# Autodesk Inventor assembly: GI - 100
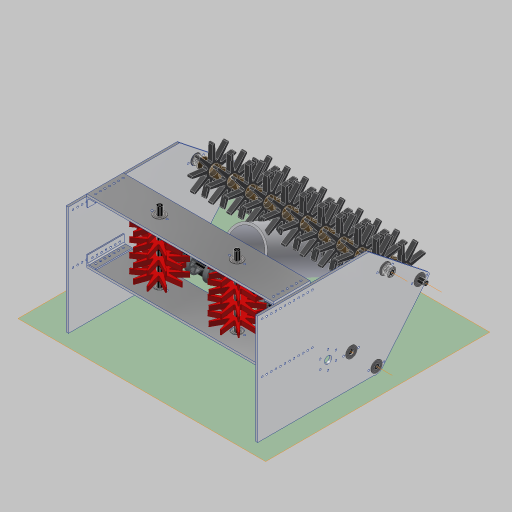
[picture p0: Inventor's stored thumbnail of the model, 512x512]
Saved by Autodesk Inventor 2023.5 (Build 275446000, 446)
## iProperties
Created: 2025-01-18
Part Number: GI - 100
Document SubType Name: Assembly
Designer: mavericks
Mass: 7269.96 g
Surface Area: 17734.9 cm^2
Volume: 4192.4 cm^3
Density: 1.73408 g/cm^3
Author: mavericks
## Documents named in this file (17)
- C:\Users\slick\OneDrive\Desktop\2025-ReefScape---CAD\ground intake\GI - 100.iam
- C:\Users\slick\OneDrive\Desktop\2025-ReefScape---CAD\ground intake\GI1\GI - 001.ipt
- C:\Users\slick\OneDrive\Desktop\2025-ReefScape---CAD\COMMON PARTS\BEARINGS\13_75mm_1_2_ThunderHex_ID_x_1_125_OD_x_0_313_WD_Flanged_Bearing_217-4006_MIR.ipt
- C:\Users\slick\OneDrive\Desktop\2025-ReefScape---CAD\ground intake\GI1\GI - 002.ipt
- C:\Users\slick\OneDrive\Desktop\2025-ReefScape---CAD\COMMON PARTS\WHEELS\2_OD_Straight_Flex_Wheel_217-6354.ipt
- C:\Users\slick\OneDrive\Desktop\2025-ReefScape---CAD\ground intake\GI - 200.iam
- C:\Users\slick\OneDrive\Desktop\2025-ReefScape---CAD\COMMON PARTS\MOTORS\Kracken with Cover and Boards.iam
- C:\Users\slick\OneDrive\Desktop\2025-ReefScape---CAD\COMMON PARTS\PULLEYS\gt2\16T Gt2 Kracken PullyWCP-1178.ipt
- C:\Users\slick\OneDrive\Desktop\2025-ReefScape---CAD\COMMON PARTS\PULLEYS\gt2\24t_x_9mm_Wide_Double_Flange_Aluminum_Pulley_GT2_3mm_1_2_Hex_Bore_217-5875.ipt
- C:\Users\slick\OneDrive\Desktop\2025-ReefScape---CAD\COMMON PARTS\PULLEYS\gt2\36t_x_9mm_Wide_Double_Flange_Aluminum_Pulley_GT2_3mm_1_2_Hex_Bore_217-5873.ipt
- C:\Users\slick\OneDrive\Desktop\2025-ReefScape---CAD\ground intake\GI1\GI - 300.iam
- C:\Users\slick\OneDrive\Desktop\2025-ReefScape---CAD\COMMON PARTS\WHEELS\WCP_1in_bore_star wheelWCP-0406.ipt
- C:\Users\slick\OneDrive\Desktop\2025-ReefScape---CAD\Field Items\Game Pieces\GE-25500.ipt
- C:\Users\slick\OneDrive\Desktop\2025-ReefScape---CAD\ground intake\GI1\GI - 007.ipt
- C:\Users\slick\OneDrive\Desktop\2025-ReefScape---CAD\ground intake\GI1\GI - 008.ipt
- C:\Users\slick\OneDrive\Desktop\2025-ReefScape---CAD\ground intake\GI1\GI - 009.ipt
- C:\Users\slick\OneDrive\Desktop\2025-ReefScape---CAD\COMMON PARTS\WHEELS\am-0619a .425 Hex Entrapption Star REV2.ipt
## Components (73 placed, 16 different names)
1. GI - 001:1 — Insert:1, Insert:2, Insert:3, Insert:4, Mate:6, Insert:18, Mate:7, Mate:15, Flush:10, Flush:11, Mate:42, Mate:43, Flush:13, Mate:45, Mate:46, Flush:17
2. 13_75mm_1_2_ThunderHex_ID_x_1_125_OD_x_0_313_WD_Flanged_Bearing_217-4006_MIR:1 — Insert:2, Mate:15, Mate:25, Mate:26
3. 13_75mm_1_2_ThunderHex_ID_x_1_125_OD_x_0_313_WD_Flanged_Bearing_217-4006_MIR:2 — Insert:1, Mate:23, Mate:24
4. 13_75mm_1_2_ThunderHex_ID_x_1_125_OD_x_0_313_WD_Flanged_Bearing_217-4006_MIR:3 — Insert:4, Mate:36
5. 13_75mm_1_2_ThunderHex_ID_x_1_125_OD_x_0_313_WD_Flanged_Bearing_217-4006_MIR:4 — Insert:3, Mate:5, Mate:10, Mate:11, Mate:12, Mate:20, Mate:21
6. GI - 001:2 — Insert:5, Insert:6, Insert:7, Insert:8, Flush:10, Mate:37, Flush:11, Insert:31, Insert:32, Insert:33, Insert:34
7. 13_75mm_1_2_ThunderHex_ID_x_1_125_OD_x_0_313_WD_Flanged_Bearing_217-4006_MIR:5 — Insert:5, Mate:33
8. 13_75mm_1_2_ThunderHex_ID_x_1_125_OD_x_0_313_WD_Flanged_Bearing_217-4006_MIR:6 — Insert:6, Mate:38, Mate:39
9. 13_75mm_1_2_ThunderHex_ID_x_1_125_OD_x_0_313_WD_Flanged_Bearing_217-4006_MIR:7 — Insert:8, Insert:16, Mate:14
10. 13_75mm_1_2_ThunderHex_ID_x_1_125_OD_x_0_313_WD_Flanged_Bearing_217-4006_MIR:8 — Insert:7
11. GI - 002:2 — Mate:17, Flush:3, Mate:20, Mate:21
12. GI - 200:1 [sub-assembly] — Insert:16, Mate:13, Mate:36
13. Kracken with Cover and Boards:1 [sub-assembly] — Insert:18, Mate:7, Mate:8, Mate:9
14. 16T Gt2 Kracken PullyWCP-1178:1 — Mate:8, Mate:9
15. 24t_x_9mm_Wide_Double_Flange_Aluminum_Pulley_GT2_3mm_1_2_Hex_Bore_217-5875:1 — Mate:10, Flush:1
16. 36t_x_9mm_Wide_Double_Flange_Aluminum_Pulley_GT2_3mm_1_2_Hex_Bore_217-5873:1 — Mate:11, Mate:12
17. 24t_x_9mm_Wide_Double_Flange_Aluminum_Pulley_GT2_3mm_1_2_Hex_Bore_217-5875:2 — Mate:13, Mate:14, Flush:1
18. 24t_x_9mm_Wide_Double_Flange_Aluminum_Pulley_GT2_3mm_1_2_Hex_Bore_217-5875:3 — Mate:17, Flush:3
19. 24t_x_9mm_Wide_Double_Flange_Aluminum_Pulley_GT2_3mm_1_2_Hex_Bore_217-5875:4 — Mate:44, Flush:12
20. 24t_x_9mm_Wide_Double_Flange_Aluminum_Pulley_GT2_3mm_1_2_Hex_Bore_217-5875:5 — Mate:23, Mate:24
21. 24t_x_9mm_Wide_Double_Flange_Aluminum_Pulley_GT2_3mm_1_2_Hex_Bore_217-5875:6 — Mate:25, Mate:26
22. GI - 300:1 [sub-assembly] — Mate:33, Mate:37, Mate:41
23. GI - 300:2 [sub-assembly] — Mate:38, Mate:39, Mate:40, Mate:44, Flush:12
24. GE-25500:1 — Tangent:1
25. GI - 007:1 — Mate:45, Flush:16, Insert:21, Insert:22, Insert:25, Insert:26, Flush:17, Insert:27, Insert:28, Mate:51
26. GI - 007:2 — Flush:16, Mate:46, Insert:19, Insert:20, Insert:23, Insert:24, Insert:29, Insert:30
27. GI - 008:1 — Insert:23, Insert:24, Insert:33, Insert:34
28. GI - 008:2 — Insert:25, Insert:26, Insert:31, Insert:32
29. GI - 008:3 — Insert:21, Insert:22
30. GI - 008:4 — Insert:19, Insert:20
31. 13_75mm_1_2_ThunderHex_ID_x_1_125_OD_x_0_313_WD_Flanged_Bearing_217-4006_MIR:9 — Insert:27, Mate:48
32. 13_75mm_1_2_ThunderHex_ID_x_1_125_OD_x_0_313_WD_Flanged_Bearing_217-4006_MIR:10 — Insert:29, Flush:18
33. 13_75mm_1_2_ThunderHex_ID_x_1_125_OD_x_0_313_WD_Flanged_Bearing_217-4006_MIR:11 — Insert:28, Mate:47
34. 13_75mm_1_2_ThunderHex_ID_x_1_125_OD_x_0_313_WD_Flanged_Bearing_217-4006_MIR:12 — Insert:30, Flush:19
35. GI - 009:1 — Mate:48, Flush:19, Mate:49
36. GI - 009:2 — Mate:47, Flush:18, Mate:50
37. 2_OD_Straight_Flex_Wheel_217-6354:1 — Mate:5, Mate:6
38. 2_OD_Straight_Flex_Wheel_217-6354:2
39. 2_OD_Straight_Flex_Wheel_217-6354:3
40. 2_OD_Straight_Flex_Wheel_217-6354:4
41. 2_OD_Straight_Flex_Wheel_217-6354:5
42. 2_OD_Straight_Flex_Wheel_217-6354:6
43. 2_OD_Straight_Flex_Wheel_217-6354:7
44. 2_OD_Straight_Flex_Wheel_217-6354:8
45. 2_OD_Straight_Flex_Wheel_217-6354:9 — Tangent:1
46. 2_OD_Straight_Flex_Wheel_217-6354:10
47. WCP_1in_bore_star wheelWCP-0406:1 — Mate:40, Mate:42
48. WCP_1in_bore_star wheelWCP-0406:3
49. WCP_1in_bore_star wheelWCP-0406:4
50. WCP_1in_bore_star wheelWCP-0406:5
51. WCP_1in_bore_star wheelWCP-0406:6
52. WCP_1in_bore_star wheelWCP-0406:7
53. WCP_1in_bore_star wheelWCP-0406:8
54. WCP_1in_bore_star wheelWCP-0406:9
55. WCP_1in_bore_star wheelWCP-0406:10
56. WCP_1in_bore_star wheelWCP-0406:11
57. WCP_1in_bore_star wheelWCP-0406:2 — Mate:41, Mate:43
58. WCP_1in_bore_star wheelWCP-0406:12
59. WCP_1in_bore_star wheelWCP-0406:13
60. WCP_1in_bore_star wheelWCP-0406:14
61. WCP_1in_bore_star wheelWCP-0406:15
62. WCP_1in_bore_star wheelWCP-0406:16
63. WCP_1in_bore_star wheelWCP-0406:17
64. WCP_1in_bore_star wheelWCP-0406:18
65. WCP_1in_bore_star wheelWCP-0406:19
66. am-0619a .425 Hex Entrapption Star REV2:2 — Mate:50, Flush:20, Mate:51
67. am-0619a .425 Hex Entrapption Star REV2:1 — Mate:49, Flush:20
68. am-0619a .425 Hex Entrapption Star REV2:3
69. am-0619a .425 Hex Entrapption Star REV2:4
70. am-0619a .425 Hex Entrapption Star REV2:5
71. am-0619a .425 Hex Entrapption Star REV2:6
72. am-0619a .425 Hex Entrapption Star REV2:7
73. am-0619a .425 Hex Entrapption Star REV2:8
## Component patterns: (10 elements, first: 2_OD_Straight_Flex_Wheel_217-6354:1), (10 elements, first: WCP_1in_bore_star wheelWCP-0406:1), (9 elements, first: WCP_1in_bore_star wheelWCP-0406:2), (4 elements, first: am-0619a .425 Hex Entrapption Star REV2:2 + am-0619a .425 Hex Entrapption Star REV2:1)
## Relationships (73: Mate 35, Insert 26, Flush 11, Tangent 1)
- Insert:1: GI - 001:1 ↔ 13_75mm_1_2_ThunderHex_ID_x_1_125_OD_x_0_313_WD_Flanged_Bearing_217-4006_MIR:2
- Insert:2: GI - 001:1 ↔ 13_75mm_1_2_ThunderHex_ID_x_1_125_OD_x_0_313_WD_Flanged_Bearing_217-4006_MIR:1
- Insert:3: GI - 001:1 ↔ 13_75mm_1_2_ThunderHex_ID_x_1_125_OD_x_0_313_WD_Flanged_Bearing_217-4006_MIR:4
- Insert:4: GI - 001:1 ↔ 13_75mm_1_2_ThunderHex_ID_x_1_125_OD_x_0_313_WD_Flanged_Bearing_217-4006_MIR:3
- Insert:5: GI - 001:2 ↔ 13_75mm_1_2_ThunderHex_ID_x_1_125_OD_x_0_313_WD_Flanged_Bearing_217-4006_MIR:5
- Insert:6: GI - 001:2 ↔ 13_75mm_1_2_ThunderHex_ID_x_1_125_OD_x_0_313_WD_Flanged_Bearing_217-4006_MIR:6
- Insert:7: GI - 001:2 ↔ 13_75mm_1_2_ThunderHex_ID_x_1_125_OD_x_0_313_WD_Flanged_Bearing_217-4006_MIR:8
- Insert:8: GI - 001:2 ↔ 13_75mm_1_2_ThunderHex_ID_x_1_125_OD_x_0_313_WD_Flanged_Bearing_217-4006_MIR:7
- Mate:5: 13_75mm_1_2_ThunderHex_ID_x_1_125_OD_x_0_313_WD_Flanged_Bearing_217-4006_MIR:4 ↔ 2_OD_Straight_Flex_Wheel_217-6354:1
- Mate:6 (36.5125 mm): GI - 001:1 ↔ 2_OD_Straight_Flex_Wheel_217-6354:1
- Insert:16: 13_75mm_1_2_ThunderHex_ID_x_1_125_OD_x_0_313_WD_Flanged_Bearing_217-4006_MIR:7 ↔ GI - 200:1
- Insert:18: GI - 001:1 ↔ Kracken with Cover and Boards:1
- Mate:7: GI - 001:1 ↔ Kracken with Cover and Boards:1
- Mate:8: Kracken with Cover and Boards:1 ↔ 16T Gt2 Kracken PullyWCP-1178:1
- Mate:9 (3.175 mm): Kracken with Cover and Boards:1 ↔ 16T Gt2 Kracken PullyWCP-1178:1
- Mate:10: 13_75mm_1_2_ThunderHex_ID_x_1_125_OD_x_0_313_WD_Flanged_Bearing_217-4006_MIR:4 ↔ 24t_x_9mm_Wide_Double_Flange_Aluminum_Pulley_GT2_3mm_1_2_Hex_Bore_217-5875:1
- Mate:11: 13_75mm_1_2_ThunderHex_ID_x_1_125_OD_x_0_313_WD_Flanged_Bearing_217-4006_MIR:4 ↔ 36t_x_9mm_Wide_Double_Flange_Aluminum_Pulley_GT2_3mm_1_2_Hex_Bore_217-5873:1
- Mate:12 (3.175 mm): 13_75mm_1_2_ThunderHex_ID_x_1_125_OD_x_0_313_WD_Flanged_Bearing_217-4006_MIR:4 ↔ 36t_x_9mm_Wide_Double_Flange_Aluminum_Pulley_GT2_3mm_1_2_Hex_Bore_217-5873:1
- Mate:13: GI - 200:1 ↔ 24t_x_9mm_Wide_Double_Flange_Aluminum_Pulley_GT2_3mm_1_2_Hex_Bore_217-5875:2
- Mate:14: 13_75mm_1_2_ThunderHex_ID_x_1_125_OD_x_0_313_WD_Flanged_Bearing_217-4006_MIR:7 ↔ 24t_x_9mm_Wide_Double_Flange_Aluminum_Pulley_GT2_3mm_1_2_Hex_Bore_217-5875:2
- Flush:1: 24t_x_9mm_Wide_Double_Flange_Aluminum_Pulley_GT2_3mm_1_2_Hex_Bore_217-5875:1 ↔ 24t_x_9mm_Wide_Double_Flange_Aluminum_Pulley_GT2_3mm_1_2_Hex_Bore_217-5875:2
- Mate:15: GI - 001:1 ↔ 13_75mm_1_2_ThunderHex_ID_x_1_125_OD_x_0_313_WD_Flanged_Bearing_217-4006_MIR:1
- Mate:17: GI - 002:2 ↔ 24t_x_9mm_Wide_Double_Flange_Aluminum_Pulley_GT2_3mm_1_2_Hex_Bore_217-5875:3
- Flush:3: GI - 002:2 ↔ 24t_x_9mm_Wide_Double_Flange_Aluminum_Pulley_GT2_3mm_1_2_Hex_Bore_217-5875:3
- Mate:20: 13_75mm_1_2_ThunderHex_ID_x_1_125_OD_x_0_313_WD_Flanged_Bearing_217-4006_MIR:4 ↔ GI - 002:2
- Mate:21: 13_75mm_1_2_ThunderHex_ID_x_1_125_OD_x_0_313_WD_Flanged_Bearing_217-4006_MIR:4 ↔ GI - 002:2
- Mate:23: 13_75mm_1_2_ThunderHex_ID_x_1_125_OD_x_0_313_WD_Flanged_Bearing_217-4006_MIR:2 ↔ 24t_x_9mm_Wide_Double_Flange_Aluminum_Pulley_GT2_3mm_1_2_Hex_Bore_217-5875:5
- Mate:24 (3.175 mm): 13_75mm_1_2_ThunderHex_ID_x_1_125_OD_x_0_313_WD_Flanged_Bearing_217-4006_MIR:2 ↔ 24t_x_9mm_Wide_Double_Flange_Aluminum_Pulley_GT2_3mm_1_2_Hex_Bore_217-5875:5
- Mate:25: 13_75mm_1_2_ThunderHex_ID_x_1_125_OD_x_0_313_WD_Flanged_Bearing_217-4006_MIR:1 ↔ 24t_x_9mm_Wide_Double_Flange_Aluminum_Pulley_GT2_3mm_1_2_Hex_Bore_217-5875:6
- Mate:26 (3.175 mm): 13_75mm_1_2_ThunderHex_ID_x_1_125_OD_x_0_313_WD_Flanged_Bearing_217-4006_MIR:1 ↔ 24t_x_9mm_Wide_Double_Flange_Aluminum_Pulley_GT2_3mm_1_2_Hex_Bore_217-5875:6
- Mate:33: 13_75mm_1_2_ThunderHex_ID_x_1_125_OD_x_0_313_WD_Flanged_Bearing_217-4006_MIR:5 ↔ GI - 300:1
- Flush:10: GI - 001:1 ↔ GI - 001:2
- Mate:36: 13_75mm_1_2_ThunderHex_ID_x_1_125_OD_x_0_313_WD_Flanged_Bearing_217-4006_MIR:3 ↔ GI - 200:1
- Mate:37: GI - 001:2 ↔ GI - 300:1
- Mate:38: 13_75mm_1_2_ThunderHex_ID_x_1_125_OD_x_0_313_WD_Flanged_Bearing_217-4006_MIR:6 ↔ GI - 300:2
- Mate:39: 13_75mm_1_2_ThunderHex_ID_x_1_125_OD_x_0_313_WD_Flanged_Bearing_217-4006_MIR:6 ↔ GI - 300:2
- Flush:11: GI - 001:1 ↔ GI - 001:2
- Mate:40: GI - 300:2 ↔ WCP_1in_bore_star wheelWCP-0406:1
- Mate:41: GI - 300:1 ↔ WCP_1in_bore_star wheelWCP-0406:2
- Mate:42 (38.1 mm): GI - 001:1 ↔ WCP_1in_bore_star wheelWCP-0406:1
- Mate:43 (63.5 mm): GI - 001:1 ↔ WCP_1in_bore_star wheelWCP-0406:2
- Mate:44: 24t_x_9mm_Wide_Double_Flange_Aluminum_Pulley_GT2_3mm_1_2_Hex_Bore_217-5875:4 ↔ GI - 300:2
- Flush:12: 24t_x_9mm_Wide_Double_Flange_Aluminum_Pulley_GT2_3mm_1_2_Hex_Bore_217-5875:4 ↔ GI - 300:2
- Tangent:1: GE-25500:1 ↔ 2_OD_Straight_Flex_Wheel_217-6354:9
- Flush:13 (6.35 mm): GI - 001:1
- Mate:45: GI - 001:1 ↔ GI - 007:1
- Flush:16: GI - 007:1 ↔ GI - 007:2
- Mate:46: GI - 001:1 ↔ GI - 007:2
- Insert:19: GI - 007:2 ↔ GI - 008:4
- Insert:20: GI - 007:2 ↔ GI - 008:4
- Insert:21: GI - 007:1 ↔ GI - 008:3
- Insert:22: GI - 007:1 ↔ GI - 008:3
- Insert:23: GI - 007:2 ↔ GI - 008:1
- Insert:24: GI - 007:2 ↔ GI - 008:1
- Insert:25: GI - 007:1 ↔ GI - 008:2
- Insert:26: GI - 007:1 ↔ GI - 008:2
- Flush:17 (50.8 mm): GI - 001:1 ↔ GI - 007:1
- Insert:27: GI - 007:1 ↔ 13_75mm_1_2_ThunderHex_ID_x_1_125_OD_x_0_313_WD_Flanged_Bearing_217-4006_MIR:9
- Insert:28: GI - 007:1 ↔ 13_75mm_1_2_ThunderHex_ID_x_1_125_OD_x_0_313_WD_Flanged_Bearing_217-4006_MIR:11
- Insert:29: GI - 007:2 ↔ 13_75mm_1_2_ThunderHex_ID_x_1_125_OD_x_0_313_WD_Flanged_Bearing_217-4006_MIR:10
- Insert:30: GI - 007:2 ↔ 13_75mm_1_2_ThunderHex_ID_x_1_125_OD_x_0_313_WD_Flanged_Bearing_217-4006_MIR:12
- Mate:47: 13_75mm_1_2_ThunderHex_ID_x_1_125_OD_x_0_313_WD_Flanged_Bearing_217-4006_MIR:11 ↔ GI - 009:2
- Flush:18: 13_75mm_1_2_ThunderHex_ID_x_1_125_OD_x_0_313_WD_Flanged_Bearing_217-4006_MIR:10 ↔ GI - 009:2
- Mate:48: 13_75mm_1_2_ThunderHex_ID_x_1_125_OD_x_0_313_WD_Flanged_Bearing_217-4006_MIR:9 ↔ GI - 009:1
- Flush:19: 13_75mm_1_2_ThunderHex_ID_x_1_125_OD_x_0_313_WD_Flanged_Bearing_217-4006_MIR:12 ↔ GI - 009:1
- Insert:31: GI - 001:2 ↔ GI - 008:2
- Insert:32: GI - 001:2 ↔ GI - 008:2
- Insert:33: GI - 001:2 ↔ GI - 008:1
- Insert:34: GI - 001:2 ↔ GI - 008:1
- Mate:49: GI - 009:1 ↔ am-0619a .425 Hex Entrapption Star REV2:1
- Mate:50: GI - 009:2 ↔ am-0619a .425 Hex Entrapption Star REV2:2
- Flush:20: am-0619a .425 Hex Entrapption Star REV2:2 ↔ am-0619a .425 Hex Entrapption Star REV2:1
- Mate:51 (12.7 mm): GI - 007:1 ↔ am-0619a .425 Hex Entrapption Star REV2:2
